# Autodesk Inventor assembly: AssemblyGripper
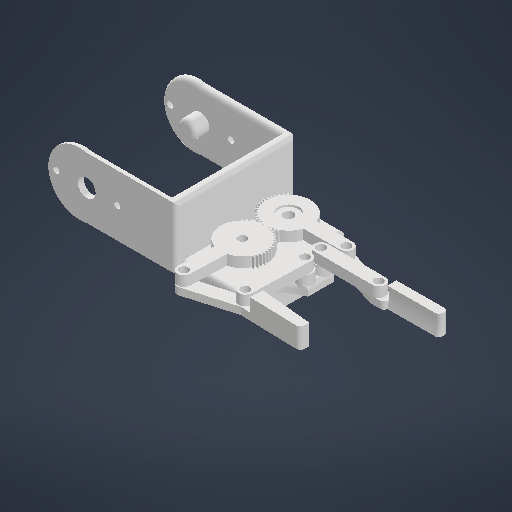
[picture p0: Inventor's stored thumbnail of the model, 512x512]
Saved by Autodesk Inventor 2026.2 (Build 302298000, 298)
## iProperties
Created: 2026-04-07
Part Number: AssemblyGripper
Document SubType Name: Assembly
Designer: Brian Wang
Author: Brian Wang
## Documents named in this file (9)
- C:\Users\Brian Wang\Downloads\RoboticsChess\3D_Model\gripper\AssemblyGripper.iam
- C:\Users\Brian Wang\Downloads\RoboticsChess\3D_Model\gripper\innerGearL.ipt
- C:\Users\Brian Wang\Downloads\RoboticsChess\3D_Model\gripper\innerGearR.ipt
- C:\Users\Brian Wang\Downloads\RoboticsChess\3D_Model\gripper\main.ipt
- C:\Users\Brian Wang\Downloads\RoboticsChess\3D_Model\gripper\testingservo.ipt
- C:\Users\Brian Wang\Downloads\RoboticsChess\3D_Model\gripper\gripsR.ipt
- C:\Users\Brian Wang\Downloads\RoboticsChess\3D_Model\gripper\innerBarR.ipt
- C:\Users\Brian Wang\Downloads\RoboticsChess\3D_Model\gripper\innerBarL.ipt
- C:\Users\Brian Wang\Downloads\RoboticsChess\3D_Model\gripper\gripsL.ipt
## Components (8 placed, 8 different names)
1. main:1 — Mate:1, Mate:2, Mate:3, Cylindrical:1, Cylindrical:3, Cylindrical:4
2. testingservo:1 — Mate:1, Mate:2, Mate:3, Cylindrical:2
3. innerGearL:1 — Cylindrical:1, Cylindrical:5
4. innerGearR:1 — Cylindrical:2, Cylindrical:6
5. gripsR:1 — Cylindrical:6, Rotational:1
6. innerBarR:1 — Cylindrical:3, Rotational:1
7. innerBarL:1 — Cylindrical:4, Rigid:1
8. gripsL:1 — Cylindrical:5, Rigid:1
## Relationships (11: CylindricalJoint 6, Mate 3, WeldJoint 1, RevoluteJoint 1)
- Mate:1: main:1 ↔ testingservo:1
- Mate:2: main:1 ↔ testingservo:1
- Mate:3: main:1 ↔ testingservo:1
- Cylindrical:1: main:1 ↔ innerGearL:1
- Cylindrical:2: testingservo:1 ↔ innerGearR:1
- Cylindrical:3: main:1 ↔ innerBarR:1
- Cylindrical:4: main:1 ↔ innerBarL:1
- Cylindrical:5: innerGearL:1 ↔ gripsL:1
- Rigid:1 [WeldJoint] (0.5 mm): innerBarL:1 ↔ gripsL:1
- Cylindrical:6: innerGearR:1 ↔ gripsR:1
- Rotational:1 [RevoluteJoint]: gripsR:1 ↔ innerBarR:1
